# Autodesk Inventor assembly: flska och kork
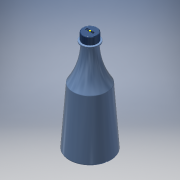
[picture p0: Inventor's stored thumbnail of the model, 180x180]
Saved by Autodesk Inventor 2018 (Build 220112000, 112)
## iProperties
Created: 2018-06-16
Part Number: flska och kork
Document SubType Name: Assembly
Designer: dilan haddad
Author: dilan haddad
## Documents named in this file (3)
- C:\Users\usr\Documents\inventor dilan\flska och kork.iam
- C:\Users\usr\Documents\inventor dilan\flaska.ipt
- C:\Users\usr\Documents\inventor dilan\kork 32.ipt
## Components (2 placed, 2 different names)
1. flaska:1 — Cylindrical:1
2. kork 32:1 — Cylindrical:1
## Relationships (1: CylindricalJoint 1)
- Cylindrical:1: flaska:1 ↔ kork 32:1
